# Autodesk Inventor assembly: Flexiwheel with Hub
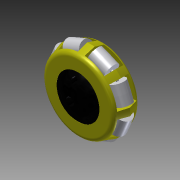
[picture p0: Inventor's stored thumbnail of the model, 180x180]
Saved by Autodesk Inventor 2014 (Build 180170000, 170)
## iProperties
Created: 2014-02-14
Part Number: Flexiwheel with Hub
Document SubType Name: Assembly
Designer: Spooner
Author: Spooner
## Documents named in this file (4)
- C:\Users\Spooner\Documents\Inventor\FerretBall Robot\3Pod\Inventor 2014 Files\Flexiwheel with Hub.iam
- C:\Users\Spooner\Documents\Inventor\FerretBall Robot\3Pod\Inventor 2014 Files\Flexiwheel Hub - Motor Side.ipt
- C:\Users\Spooner\Documents\Inventor\FerretBall Robot\3Pod\Inventor 2014 Files\Flexiwheel Hub - Out Side.ipt
- C:\Users\Spooner\Documents\Inventor\FerretBall Robot\3Pod\Inventor 2014 Files\Flexiwheel.iam
## Components (3 placed, 3 different names)
1. Flexiwheel Hub - Motor Side:1 — Insert:2, Mate:2
2. Flexiwheel Hub - Out Side:1 — Insert:1, Mate:1
3. Flexiwheel:1 [sub-assembly] — Insert:1, Mate:1, Insert:2, Mate:2
## Relationships (4: Insert 2, Mate 2)
- Insert:1: Flexiwheel Hub - Out Side:1 ↔ Flexiwheel:1
- Mate:1: Flexiwheel Hub - Out Side:1 ↔ Flexiwheel:1
- Insert:2: Flexiwheel Hub - Motor Side:1 ↔ Flexiwheel:1
- Mate:2: Flexiwheel Hub - Motor Side:1 ↔ Flexiwheel:1
